# Autodesk Inventor assembly: 3D_PrintParts_1
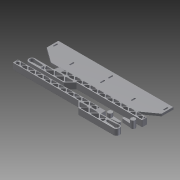
[picture p0: Inventor's stored thumbnail of the model, 180x180]
Saved by Autodesk Inventor 2011 SP2 (Build 150309200, 309)
## iProperties
Created: 2015-11-08
Part Number: 3D_PrintParts_1
Document SubType Name: Assembly
Designer: Ernest
Author: Ernest
## Documents named in this file (5)
- D:\Inventor\Sumobot_3rd_Year\3D_Print_Parts_1.iam
- D:\Inventor\Sumobot_3rd_Year\Front_Plate.ipt
- D:\Inventor\Sumobot_3rd_Year\Robot_ARM_Pivot.ipt
- D:\Inventor\Sumobot_3rd_Year\Robot_ARM_LEFT.ipt
- D:\Inventor\Sumobot_3rd_Year\Robot_ARM_RIGHT.ipt
## Components (5 placed, 4 different names)
1. Front_Plate:1 — Mate:3, Mate:5, Flush:3, Flush:4
2. Robot_ARM_Pivot:1 — Flush:2
3. Robot_ARM_Pivot:2 — Flush:2, Mate:4
4. Robot_ARM_LEFT:1 — Flush:1, Mate:1, Mate:2, Mate:6, Flush:3
5. Robot_ARM_RIGHT:1 — Flush:1, Mate:5, Mate:6, Flush:4
## Relationships (10: Mate 6, Flush 4)
- Flush:1: Robot_ARM_LEFT:1 ↔ Robot_ARM_RIGHT:1
- Mate:1: Robot_ARM_LEFT:1
- Mate:2: Robot_ARM_LEFT:1
- Mate:3: Front_Plate:1
- Flush:2: Robot_ARM_Pivot:1 ↔ Robot_ARM_Pivot:2
- Mate:4: Robot_ARM_Pivot:2
- Mate:5 (5 mm): Front_Plate:1 ↔ Robot_ARM_RIGHT:1
- Mate:6 (5 mm): Robot_ARM_LEFT:1 ↔ Robot_ARM_RIGHT:1
- Flush:3: Front_Plate:1 ↔ Robot_ARM_LEFT:1
- Flush:4: Front_Plate:1 ↔ Robot_ARM_RIGHT:1
